# Autodesk Inventor assembly: Right side arm
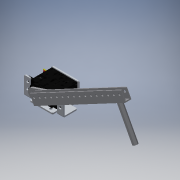
[picture p0: Inventor's stored thumbnail of the model, 180x180]
Saved by Autodesk Inventor 2019 (Build 230136000, 136)
## iProperties
Created: 2020-02-15
Part Number: Right side arm
Document SubType Name: Assembly
Designer: Delta
Author: Delta
## Documents named in this file (6)
- C:\Robotics\2019-20_CAD\Drive Train\Right side arm.iam
- C:\Robotics\COTSParts\Tetrix\39060_txm-standard servo bracket.ipt
- C:\Robotics\COTSParts\Tetrix\Tetrix 180 Servo.ipt
- C:\Robotics\2019-20_CAD\Collection\Servo horn.ipt
- C:\Robotics\2019-20_CAD\Drive Train\585392MiniChannel6.31in.ipt
- C:\Robotics\COTSParts\Tetrix\Hex standoff 2in.ipt
## Components (5 placed, 5 different names)
1. 39060_txm-standard servo bracket:1 — Mate:9, Angle:3, Mate:10
2. Tetrix 180 Servo:1 — Mate:9, Angle:3, Mate:10, Mate:13, Mate:14
3. Servo horn:1 — Mate:11, Mate:12, Angle:4, Mate:13, Mate:14
4. 585392MiniChannel6.31in:1 — Mate:7, Mate:8, Mate:11, Mate:12, Angle:4
5. Hex standoff 2in:1 — Mate:7, Mate:8
## Relationships (10: Mate 8, Angle 2)
- Mate:7: 585392MiniChannel6.31in:1 ↔ Hex standoff 2in:1
- Mate:8: 585392MiniChannel6.31in:1 ↔ Hex standoff 2in:1
- Mate:9: 39060_txm-standard servo bracket:1 ↔ Tetrix 180 Servo:1
- Angle:3 (0 deg): 39060_txm-standard servo bracket:1 ↔ Tetrix 180 Servo:1
- Mate:10: 39060_txm-standard servo bracket:1 ↔ Tetrix 180 Servo:1
- Mate:11: Servo horn:1 ↔ 585392MiniChannel6.31in:1
- Mate:12: Servo horn:1 ↔ 585392MiniChannel6.31in:1
- Angle:4 (5 deg): Servo horn:1 ↔ 585392MiniChannel6.31in:1
- Mate:13: Tetrix 180 Servo:1 ↔ Servo horn:1
- Mate:14: Tetrix 180 Servo:1 ↔ Servo horn:1
